# Autodesk Inventor assembly: SHOT_1_002_ShooterAssembly
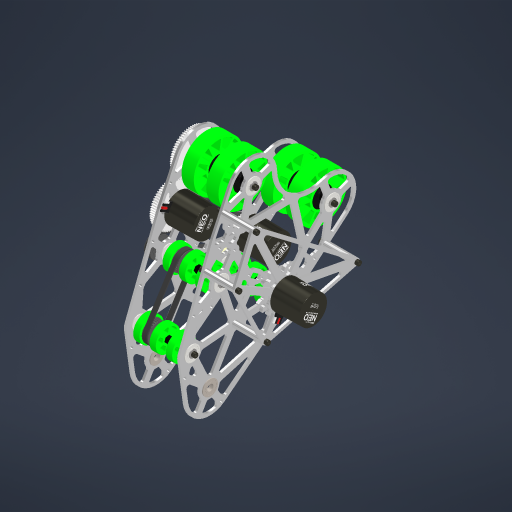
[picture p0: Inventor's stored thumbnail of the model, 512x512]
Saved by Autodesk Inventor 2024.2 (Build 282272000, 272)
## iProperties
Created: 2024-08-07
Part Number: SHOT_1_002_ShooterAssembly
Document SubType Name: Assembly
Designer: Kenji
Mass: 3332.01 g
Surface Area: 7576.03 cm^2
Volume: 1529.69 cm^3
Density: 2.17823 g/cm^3
Author: Kenji
## Documents named in this file (34)
- C:\Users\bobsb\OneDrive\Documents\GitHub\1622-2024-Summer-CAD-A-Thon\Shooter\SHOT_1_002_ShooterAssembly.iam
- C:\Users\bobsb\OneDrive\Documents\GitHub\1622-2024-Summer-CAD-A-Thon\Shooter\SHOT_1_001_ShooterPlate.ipt
- C:\Users\bobsb\OneDrive\Documents\GitHub\1622-2024-Summer-CAD-A-Thon\COTS Library\Motion\Wheels\Compliant Wheels\4in compliant wheels\0.500in hex bore\COTS_am-3462_4indiameter_0.500inhexbore_durometer35A_CompliantWheel.ipt
- C:\Users\bobsb\OneDrive\Documents\GitHub\1622-2024-Summer-CAD-A-Thon\COTS Library\Motion\Bearings\COTS_WCP-0783_1.125ODHexBearing.ipt
- C:\Users\bobsb\OneDrive\Documents\GitHub\1622-2024-Summer-CAD-A-Thon\COTS Library\Motion\Bearings\COTS_WCP-0781_0.5ODCircularFlangedBearing.ipt
- C:\Users\bobsb\OneDrive\Documents\GitHub\1622-2024-Summer-CAD-A-Thon\COTS Library\Motors\COTS_REV-21-1650-V1.1_Neo1.1.ipt
- C:\Users\bobsb\OneDrive\Documents\GitHub\1622-2024-Summer-CAD-A-Thon\COTS Library\Motion\Wheels\Compliant Wheels\2in compliant wheels\0.500in hex bore\COTS_am-3462_2indiameter_0.500inhexbore_durometer35A_CompliantWheel.ipt
- C:\Users\bobsb\OneDrive\Documents\GitHub\1622-2024-Summer-CAD-A-Thon\COTS Library\Fasteners\Bolts\Button-Head\10-32\COTS_92949A265_1-2in long Stainless Steel Button Head Screw.ipt
- C:\Users\bobsb\OneDrive\Documents\GitHub\1622-2024-Summer-CAD-A-Thon\COTS Library\Motion\Pulleys\HTD5M\10mm Wide\COTS_HTD5M10mm24T_WCP-0564.ipt
- C:\Users\bobsb\OneDrive\Documents\GitHub\1622-2024-Summer-CAD-A-Thon\COTS Library\Adapters\COTS_REV-21-1879_8mmKeyTo0.5Hex.ipt
- C:\Users\bobsb\OneDrive\Documents\GitHub\1622-2024-Summer-CAD-A-Thon\COTS Library\Motion\Gears\20DP gears\Aluminum\COTS_WCP-0171_66T.ipt
- C:\Users\bobsb\OneDrive\Documents\GitHub\1622-2024-Summer-CAD-A-Thon\Shooter\SHOT_1_004_66TGear-24TPulley.ipt
- C:\Users\bobsb\OneDrive\Documents\GitHub\1622-2024-Summer-CAD-A-Thon\COTS Library\Motion\Gears\20DP gears\Aluminum\COTS_WCP-0717_54T.ipt
- C:\Users\bobsb\OneDrive\Documents\GitHub\1622-2024-Summer-CAD-A-Thon\Shooter\SHOT_1_005_36TGear-24TPulley.ipt
- C:\Users\bobsb\OneDrive\Documents\GitHub\1622-2024-Summer-CAD-A-Thon\Shooter\SHOT_1_014_Belt3.ipt
- C:\Users\bobsb\OneDrive\Documents\GitHub\1622-2024-Summer-CAD-A-Thon\Shooter\SHOT_1_013_Belt2.ipt
- C:\Users\bobsb\OneDrive\Documents\GitHub\1622-2024-Summer-CAD-A-Thon\Shooter\SHOT_1_012_Belt1.ipt
- C:\Users\bobsb\OneDrive\Documents\GitHub\1622-2024-Summer-CAD-A-Thon\Shooter\SHOT_1_010_Spacer1.ipt
- C:\Users\bobsb\OneDrive\Documents\GitHub\1622-2024-Summer-CAD-A-Thon\Shooter\SHOT_1_011_Spacer2.ipt
- C:\Users\bobsb\OneDrive\Documents\GitHub\1622-2024-Summer-CAD-A-Thon\Shooter\SHOT_1_006_HexShaft1.ipt
- C:\Users\bobsb\OneDrive\Documents\GitHub\1622-2024-Summer-CAD-A-Thon\Shooter\SHOT_1_007_HexShaft2.ipt
- C:\Users\bobsb\OneDrive\Documents\GitHub\1622-2024-Summer-CAD-A-Thon\Shooter\SHOT_1_008_HexShaft3.ipt
- C:\Users\bobsb\OneDrive\Documents\GitHub\1622-2024-Summer-CAD-A-Thon\Shooter\SHOT_1_009_HexShaft4.ipt
- C:\Users\bobsb\OneDrive\Documents\GitHub\1622-2024-Summer-CAD-A-Thon\COTS Library\Fasteners\Bolts\Socket-Head\0.25-20\COTS_91251A539_Black-Oxide Alloy Steel Socket Head Screw (1).ipt
- C:\Users\bobsb\OneDrive\Documents\GitHub\1622-2024-Summer-CAD-A-Thon\COTS Library\Fasteners\Washers\COTS_90107A029_316 Stainless Steel Washer.ipt
- C:\Users\bobsb\OneDrive\Documents\GitHub\1622-2024-Summer-CAD-A-Thon\COTS Library\Fasteners\Bolts\Button-Head\10-32\COTS_92949A267_18-8 Stainless Steel Button Head Hex Drive Screw (1).ipt
- C:\Users\bobsb\OneDrive\Documents\GitHub\1622-2024-Summer-CAD-A-Thon\COTS Library\Fasteners\Washers\COTS_91860A047_Size10Washer.ipt
- C:\Users\bobsb\OneDrive\Documents\GitHub\1622-2024-Summer-CAD-A-Thon\COTS Library\Fasteners\Shaft Collars\COTS_WCP-0799_0.5inchHexShaftCollar.ipt
- C:\Users\bobsb\OneDrive\Documents\GitHub\1622-2024-Summer-CAD-A-Thon\Shooter\SHOT_1_015_PivotCover.ipt
- C:\Users\bobsb\OneDrive\Documents\GitHub\1622-2024-Summer-CAD-A-Thon\Shooter\SHOT_1_016_5DP14TGear.ipt
- C:\Users\bobsb\OneDrive\Documents\GitHub\1622-2024-Summer-CAD-A-Thon\Shooter\SHOT_1_017_Spacer3.ipt
- C:\Users\bobsb\OneDrive\Documents\GitHub\1622-2024-Summer-CAD-A-Thon\Shooter\SHOT_1_0018_Spacer4.ipt
- C:\Users\bobsb\OneDrive\Documents\GitHub\1622-2024-Summer-CAD-A-Thon\Shooter\SHOY_019_Spacer5.ipt
- C:\Users\bobsb\OneDrive\Documents\GitHub\1622-2024-Summer-CAD-A-Thon\COTS Library\Fasteners\Bolts\Button-Head\0.25-20\COTS_0.25-20_ButtonHead_0.5inlong_StainlessSteel_92949A537.ipt
## Components (109 placed, 33 different names)
1. SHOT_1_001_ShooterPlate:1 — Mate:140, Mate:141, Mate:143, Mate:144, Mate:148, Mate:150, Mate:151, Mate:152, Mate:160, Mate:161, Mate:163, Mate:164, Mate:165, Mate:166, Mate:167, Mate:168, Mate:169, Mate:170, Mate:171, Mate:172, Mate:270, Mate:271, Mate:280, Mate:281, Mate:282, Mate:283, Mate:284, Mate:285, Mate:286, Mate:287, Mate:288, Mate:289, Mate:290, Mate:294, Mate:304, Mate:305
2. SHOT_1_001_ShooterPlate:2 — Mate:140, Mate:141, Mate:147, Mate:149, Mate:156, Mate:158, Mate:159, Mate:272, Mate:273, Mate:304, Mate:311, Mate:337, Mate:353, Mate:354, Mate:371, Mate:374, Mate:375, Mate:377, Mate:387, Mate:388, Mate:389, Mate:390, Mate:391, Mate:394, Mate:395, Mate:396, Mate:397
3. COTS_WCP-0783_1.125ODHexBearing:1 — Mate:139, Flush:5, Mate:156, Mate:246
4. COTS_WCP-0783_1.125ODHexBearing:2 — Mate:147, Mate:149, Mate:333, Mate:343
5. COTS_WCP-0783_1.125ODHexBearing:3 — Mate:36, Mate:102, Flush:5, Mate:251
6. COTS_WCP-0783_1.125ODHexBearing:5 — Mate:244, Mate:270, Mate:271, Mate:274, Mate:275
7. COTS_WCP-0783_1.125ODHexBearing:9 — Mate:102, Flush:4, Mate:150, Mate:152, Mate:186, Mate:187
8. COTS_WCP-0783_1.125ODHexBearing:10 — Mate:31, Mate:104, Flush:4, Mate:151, Mate:188, Mate:213
9. COTS_WCP-0783_1.125ODHexBearing:11 — Mate:49, Mate:52, Mate:143, Mate:144, Flush:17, Mate:346
10. COTS_WCP-0783_1.125ODHexBearing:12 — Mate:272, Mate:273, Mate:278
11. COTS_WCP-0781_0.5ODCircularFlangedBearing:1 — Mate:138, Mate:158, Mate:159
12. COTS_WCP-0781_0.5ODCircularFlangedBearing:2 — Mate:138, Mate:160
13. COTS_REV-21-1650-V1.1_Neo1.1:1 — Mate:133, Mate:161, Mate:163, Mate:185, Mate:256, Mate:260, Mate:261, Mate:266
14. COTS_92949A265_1-2in long Stainless Steel Button Head Screw:1 — Mate:165, Mate:168, Mate:185
15. COTS_92949A265_1-2in long Stainless Steel Button Head Screw:2 — Mate:167, Mate:170
16. COTS_92949A265_1-2in long Stainless Steel Button Head Screw:3 — Mate:166, Mate:169
17. COTS_92949A265_1-2in long Stainless Steel Button Head Screw:4 — Mate:164, Mate:171
18. COTS_WCP-0783_1.125ODHexBearing:13 — Mate:148, Mate:305, Mate:306, Mate:342
19. COTS_WCP-0783_1.125ODHexBearing:14 — Mate:308, Mate:311, Mate:337
20. COTS_REV-21-1650-V1.1_Neo1.1:2 — Mate:280, Mate:281, Mate:282, Mate:291, Mate:292, Mate:293, Mate:295
21. COTS_REV-21-1879_8mmKeyTo0.5Hex:1 — Mate:291, Mate:292
22. COTS_92949A265_1-2in long Stainless Steel Button Head Screw:5 — Mate:285, Mate:288
23. COTS_92949A265_1-2in long Stainless Steel Button Head Screw:6 — Mate:286, Mate:290
24. COTS_92949A265_1-2in long Stainless Steel Button Head Screw:7 — Mate:283, Mate:287
25. COTS_92949A265_1-2in long Stainless Steel Button Head Screw:8 — Mate:284, Mate:289
26. SHOT_1_004_66TGear-24TPulley:1 — Mate:133, Mate:172, Flush:6, Mate:198, Mate:257
27. COTS_WCP-0171_66T:1 — Mate:186, Mate:187, Mate:301, Flush:15
28. COTS_HTD5M10mm24T_WCP-0564:1 — Mate:188, Flush:6, Mate:199, Mate:200, Mate:207, Flush:9, Mate:214, Mate:240
29. COTS_WCP-0717_54T:1 — Mate:274, Mate:275, Mate:276, Flush:13, Mate:329, Mate:330
30. SHOT_1_005_36TGear-24TPulley:1 — Mate:293, Mate:294, Mate:296, Flush:16, Mate:318, Mate:319
31. COTS_HTD5M10mm24T_WCP-0564:2 — Mate:320, Mate:331, Mate:339, Mate:340
32. COTS_HTD5M10mm24T_WCP-0564:3 — Flush:16, Mate:307, Mate:317, Mate:326, Flush:18
33. COTS_HTD5M10mm24T_WCP-0564:4 — Mate:255, Mate:314, Mate:321, Mate:335, Mate:336, Mate:338
34. SHOT_1_014_Belt3:1 — Mate:255, Mate:320, Mate:321, Mate:331
35. SHOT_1_013_Belt2:1 — Mate:317, Mate:318, Mate:319
36. SHOT_1_012_Belt1:1 — Mate:198, Mate:199, Mate:200
37. SHOT_1_010_Spacer1:1 — Mate:213, Mate:214
38. SHOT_1_010_Spacer1:2 — Mate:306, Mate:307
39. SHOT_1_006_HexShaft1:1 — Mate:235, Mate:301, Flush:15, Mate:302, Mate:303
40. SHOT_1_007_HexShaft2:1 — Mate:207, Flush:9, Mate:238, Mate:245
41. SHOT_1_009_HexShaft4:1 — Mate:237, Mate:248, Mate:308, Flush:17, Mate:310, Mate:312
42. SHOT_1_006_HexShaft1:2 — Mate:239, Mate:249, Mate:276, Flush:13
43. COTS_91251A539_Black-Oxide Alloy Steel Socket Head Screw (1):1 — Mate:219, Mate:233, Mate:239
44. COTS_91251A539_Black-Oxide Alloy Steel Socket Head Screw (1):2 — Mate:220, Mate:230, Mate:238
45. COTS_91251A539_Black-Oxide Alloy Steel Socket Head Screw (1):3 — Mate:222, Mate:229, Mate:249
46. COTS_91251A539_Black-Oxide Alloy Steel Socket Head Screw (1):4 — Mate:217, Mate:232, Mate:303
47. COTS_91251A539_Black-Oxide Alloy Steel Socket Head Screw (1):5 — Mate:218, Mate:234, Mate:235
48. COTS_91251A539_Black-Oxide Alloy Steel Socket Head Screw (1):6 — Mate:316, Mate:324
49. COTS_91251A539_Black-Oxide Alloy Steel Socket Head Screw (1):7 — Mate:224, Mate:237, Mate:309
50. COTS_91251A539_Black-Oxide Alloy Steel Socket Head Screw (1):8 — Mate:223, Mate:227
51. COTS_91251A539_Black-Oxide Alloy Steel Socket Head Screw (1):9 — Mate:216, Mate:248, Mate:313, Mate:314
52. COTS_91251A539_Black-Oxide Alloy Steel Socket Head Screw (1):10 — Mate:215, Mate:231, Mate:245
53. COTS_90107A029_316 Stainless Steel Washer:1 — Mate:218, Mate:234, Mate:302
54. COTS_90107A029_316 Stainless Steel Washer:2 — Mate:220, Mate:230, Mate:240
55. COTS_90107A029_316 Stainless Steel Washer:3 — Mate:316, Mate:324, Mate:333
56. COTS_90107A029_316 Stainless Steel Washer:4 — Mate:219, Mate:233, Mate:244
57. COTS_90107A029_316 Stainless Steel Washer:5 — Mate:222, Mate:229, Mate:278
58. COTS_90107A029_316 Stainless Steel Washer:6 — Mate:223, Mate:227, Mate:326
59. COTS_90107A029_316 Stainless Steel Washer:7 — Mate:224, Mate:309, Mate:310
60. COTS_90107A029_316 Stainless Steel Washer:8 — Mate:217, Mate:232, Mate:251
61. COTS_90107A029_316 Stainless Steel Washer:9 — Mate:215, Mate:231, Mate:246
62. COTS_90107A029_316 Stainless Steel Washer:10 — Mate:216, Mate:312, Mate:313
63. SHOT_1_011_Spacer2:1 — Mate:256, Mate:257, Mate:267
64. SHOT_1_011_Spacer2:2 — Mate:269, Mate:279, Mate:296
65. COTS_REV-21-1879_8mmKeyTo0.5Hex:2 — Mate:260, Mate:261
66. COTS_92949A267_18-8 Stainless Steel Button Head Hex Drive Screw (1):1 — Mate:263, Mate:265, Mate:266
67. COTS_92949A267_18-8 Stainless Steel Button Head Hex Drive Screw (1):2 — Mate:262, Mate:264, Mate:279, Mate:295
68. COTS_91860A047_Size10Washer:1 — Mate:262, Mate:264, Mate:269
69. COTS_91860A047_Size10Washer:2 — Mate:263, Mate:265, Mate:267
70. COTS_90107A029_316 Stainless Steel Washer:11 — Mate:327, Mate:328, Mate:329, Mate:330
71. COTS_91251A539_Black-Oxide Alloy Steel Socket Head Screw (1):11 — Mate:327, Mate:328
72. COTS_WCP-0799_0.5inchHexShaftCollar:1 — Mate:339, Mate:340, Mate:341
73. COTS_WCP-0799_0.5inchHexShaftCollar:2 — Mate:336, Mate:338
74. COTS_WCP-0799_0.5inchHexShaftCollar:3 — Mate:344, Mate:345
75. COTS_WCP-0799_0.5inchHexShaftCollar:4 — Mate:346, Mate:347
76. SHOT_1_008_HexShaft3:1 — Mate:343, Flush:18
77. SHOT_1_015_PivotCover:3 — Mate:353, Mate:354, Mate:357, Mate:358, Mate:359, Mate:368, Mate:372, Mate:373, Mate:376, Mate:378, Mate:379, Mate:380, Mate:381, Mate:382, Mate:383, Mate:384, Mate:385, Mate:386
78. COTS_REV-21-1650-V1.1_Neo1.1:3 — Mate:357, Mate:358, Mate:359, Mate:360, Mate:361, Mate:362, Mate:367, Mate:369, Mate:398, Mate:401, Mate:402
79. COTS_REV-21-1879_8mmKeyTo0.5Hex:3 — Mate:360, Mate:361
80. COTS_92949A265_1-2in long Stainless Steel Button Head Screw:9 — Mate:362, Mate:403
81. SHOT_1_017_Spacer3:1 — Mate:367, Mate:368, Mate:399
82. SHOT_1_0018_Spacer4:1 — Mate:369, Mate:400
83. SHOY_019_Spacer5:1 — Mate:377, Mate:378
84. SHOY_019_Spacer5:2 — Mate:375, Mate:376, Mate:397
85. SHOY_019_Spacer5:3 — Mate:371, Mate:372
86. SHOY_019_Spacer5:4 — Mate:373, Mate:374
87. COTS_91251A539_Black-Oxide Alloy Steel Socket Head Screw (1):13 — Mate:382, Mate:384
88. COTS_91251A539_Black-Oxide Alloy Steel Socket Head Screw (1):14 — Mate:388, Mate:390
89. COTS_91251A539_Black-Oxide Alloy Steel Socket Head Screw (1):15 — Mate:391, Mate:394
90. COTS_91251A539_Black-Oxide Alloy Steel Socket Head Screw (1):16 — Mate:387, Mate:389
91. COTS_91251A539_Black-Oxide Alloy Steel Socket Head Screw (1):17 — Mate:379, Mate:385
92. COTS_91251A539_Black-Oxide Alloy Steel Socket Head Screw (1):18 — Mate:380, Mate:386
93. COTS_91251A539_Black-Oxide Alloy Steel Socket Head Screw (1):19 — Mate:381, Mate:383
94. COTS_0.25-20_ButtonHead_0.5inlong_StainlessSteel_92949A537:1 — Mate:395, Mate:396
95. SHOT_1_016_5DP14TGear:2 — Mate:398, Mate:399, Mate:400
96. COTS_90107A029_316 Stainless Steel Washer:12 — Mate:401, Mate:402, Mate:403
97. COTS_am-3462_4indiameter_0.500inhexbore_durometer35A_CompliantWheel:4 — Mate:36, Flush:3
98. COTS_am-3462_4indiameter_0.500inhexbore_durometer35A_CompliantWheel:1 — Mate:31, Flush:3, Mate:104
99. COTS_am-3462_4indiameter_0.500inhexbore_durometer35A_CompliantWheel:5
100. COTS_am-3462_4indiameter_0.500inhexbore_durometer35A_CompliantWheel:6 — Mate:139
101. COTS_am-3462_2indiameter_0.500inhexbore_durometer35A_CompliantWheel:1 — Flush:1, Flush:2
102. COTS_am-3462_2indiameter_0.500inhexbore_durometer35A_CompliantWheel:6 — Flush:2, Mate:341, Mate:342, Mate:344, Mate:345
103. COTS_am-3462_2indiameter_0.500inhexbore_durometer35A_CompliantWheel:2 — Mate:49, Flush:1, Mate:52, Mate:335, Mate:347
104. COTS_am-3462_2indiameter_0.500inhexbore_durometer35A_CompliantWheel:7
105. COTS_am-3462_2indiameter_0.500inhexbore_durometer35A_CompliantWheel:8
106. COTS_am-3462_2indiameter_0.500inhexbore_durometer35A_CompliantWheel:9
107. COTS_am-3462_2indiameter_0.500inhexbore_durometer35A_CompliantWheel:10
108. COTS_am-3462_2indiameter_0.500inhexbore_durometer35A_CompliantWheel:11
109. COTS_am-3462_2indiameter_0.500inhexbore_durometer35A_CompliantWheel:12
## Component patterns: (2 elements, first: COTS_am-3462_4indiameter_0.500inhexbore_durometer35A_CompliantWheel:4 + COTS_am-3462_4indiameter_0.500inhexbore_durometer35A_CompliantWheel:1), (3 elements, first: COTS_am-3462_2indiameter_0.500inhexbore_durometer35A_CompliantWheel:1 + COTS_am-3462_2indiameter_0.500inhexbore_durometer35A_CompliantWheel:6 + COTS_am-3462_2indiameter_0.500inhexbore_durometer35A_CompliantWheel:2)
## Relationships (204: Mate 192, Flush 12)
- Mate:31: COTS_WCP-0783_1.125ODHexBearing:10 ↔ COTS_am-3462_4indiameter_0.500inhexbore_durometer35A_CompliantWheel:1
- Mate:36: COTS_WCP-0783_1.125ODHexBearing:3 ↔ COTS_am-3462_4indiameter_0.500inhexbore_durometer35A_CompliantWheel:4
- Mate:49: COTS_WCP-0783_1.125ODHexBearing:11 ↔ COTS_am-3462_2indiameter_0.500inhexbore_durometer35A_CompliantWheel:2
- Flush:1: COTS_am-3462_2indiameter_0.500inhexbore_durometer35A_CompliantWheel:1 ↔ COTS_am-3462_2indiameter_0.500inhexbore_durometer35A_CompliantWheel:2
- Flush:2: COTS_am-3462_2indiameter_0.500inhexbore_durometer35A_CompliantWheel:1 ↔ COTS_am-3462_2indiameter_0.500inhexbore_durometer35A_CompliantWheel:6
- Mate:52 (12.7 mm): COTS_WCP-0783_1.125ODHexBearing:11 ↔ COTS_am-3462_2indiameter_0.500inhexbore_durometer35A_CompliantWheel:2
- Mate:102: COTS_WCP-0783_1.125ODHexBearing:3 ↔ COTS_WCP-0783_1.125ODHexBearing:9
- Flush:3: COTS_am-3462_4indiameter_0.500inhexbore_durometer35A_CompliantWheel:4 ↔ COTS_am-3462_4indiameter_0.500inhexbore_durometer35A_CompliantWheel:1
- Mate:104 (12.7 mm): COTS_WCP-0783_1.125ODHexBearing:10 ↔ COTS_am-3462_4indiameter_0.500inhexbore_durometer35A_CompliantWheel:1
- Mate:133: COTS_REV-21-1650-V1.1_Neo1.1:1 ↔ SHOT_1_004_66TGear-24TPulley:1
- Mate:138: COTS_WCP-0781_0.5ODCircularFlangedBearing:1 ↔ COTS_WCP-0781_0.5ODCircularFlangedBearing:2
- Mate:139: COTS_WCP-0783_1.125ODHexBearing:1 ↔ COTS_am-3462_4indiameter_0.500inhexbore_durometer35A_CompliantWheel:6
- Flush:4: COTS_WCP-0783_1.125ODHexBearing:9 ↔ COTS_WCP-0783_1.125ODHexBearing:10
- Flush:5: COTS_WCP-0783_1.125ODHexBearing:1 ↔ COTS_WCP-0783_1.125ODHexBearing:3
- Mate:140: SHOT_1_001_ShooterPlate:1 ↔ SHOT_1_001_ShooterPlate:2
- Mate:141: SHOT_1_001_ShooterPlate:1 ↔ SHOT_1_001_ShooterPlate:2
- Mate:143: SHOT_1_001_ShooterPlate:1 ↔ COTS_WCP-0783_1.125ODHexBearing:11
- Mate:144: SHOT_1_001_ShooterPlate:1 ↔ COTS_WCP-0783_1.125ODHexBearing:11
- Mate:147: SHOT_1_001_ShooterPlate:2 ↔ COTS_WCP-0783_1.125ODHexBearing:2
- Mate:148: SHOT_1_001_ShooterPlate:1 ↔ COTS_WCP-0783_1.125ODHexBearing:13
- Mate:149: SHOT_1_001_ShooterPlate:2 ↔ COTS_WCP-0783_1.125ODHexBearing:2
- Mate:150: SHOT_1_001_ShooterPlate:1 ↔ COTS_WCP-0783_1.125ODHexBearing:9
- Mate:151: SHOT_1_001_ShooterPlate:1 ↔ COTS_WCP-0783_1.125ODHexBearing:10
- Mate:152: SHOT_1_001_ShooterPlate:1 ↔ COTS_WCP-0783_1.125ODHexBearing:9
- Mate:156: SHOT_1_001_ShooterPlate:2 ↔ COTS_WCP-0783_1.125ODHexBearing:1
- Mate:158: SHOT_1_001_ShooterPlate:2 ↔ COTS_WCP-0781_0.5ODCircularFlangedBearing:1
- Mate:159: SHOT_1_001_ShooterPlate:2 ↔ COTS_WCP-0781_0.5ODCircularFlangedBearing:1
- Mate:160: SHOT_1_001_ShooterPlate:1 ↔ COTS_WCP-0781_0.5ODCircularFlangedBearing:2
- Mate:161: SHOT_1_001_ShooterPlate:1 ↔ COTS_REV-21-1650-V1.1_Neo1.1:1
- Mate:163: SHOT_1_001_ShooterPlate:1 ↔ COTS_REV-21-1650-V1.1_Neo1.1:1
- Mate:164: SHOT_1_001_ShooterPlate:1 ↔ COTS_92949A265_1-2in long Stainless Steel Button Head Screw:4
- Mate:165: SHOT_1_001_ShooterPlate:1 ↔ COTS_92949A265_1-2in long Stainless Steel Button Head Screw:1
- Mate:166: SHOT_1_001_ShooterPlate:1 ↔ COTS_92949A265_1-2in long Stainless Steel Button Head Screw:3
- Mate:167: SHOT_1_001_ShooterPlate:1 ↔ COTS_92949A265_1-2in long Stainless Steel Button Head Screw:2
- Mate:168: SHOT_1_001_ShooterPlate:1 ↔ COTS_92949A265_1-2in long Stainless Steel Button Head Screw:1
- Mate:169: SHOT_1_001_ShooterPlate:1 ↔ COTS_92949A265_1-2in long Stainless Steel Button Head Screw:3
- Mate:170: SHOT_1_001_ShooterPlate:1 ↔ COTS_92949A265_1-2in long Stainless Steel Button Head Screw:2
- Mate:171: SHOT_1_001_ShooterPlate:1 ↔ COTS_92949A265_1-2in long Stainless Steel Button Head Screw:4
- Mate:172: SHOT_1_001_ShooterPlate:1 ↔ SHOT_1_004_66TGear-24TPulley:1
- Mate:185: COTS_REV-21-1650-V1.1_Neo1.1:1 ↔ COTS_92949A265_1-2in long Stainless Steel Button Head Screw:1
- Mate:186: COTS_WCP-0783_1.125ODHexBearing:9 ↔ COTS_WCP-0171_66T:1
- Mate:187: COTS_WCP-0783_1.125ODHexBearing:9 ↔ COTS_WCP-0171_66T:1
- Mate:188: COTS_WCP-0783_1.125ODHexBearing:10 ↔ COTS_HTD5M10mm24T_WCP-0564:1
- Flush:6: SHOT_1_004_66TGear-24TPulley:1 ↔ COTS_HTD5M10mm24T_WCP-0564:1
- Mate:198: SHOT_1_004_66TGear-24TPulley:1 ↔ SHOT_1_012_Belt1:1
- Mate:199: COTS_HTD5M10mm24T_WCP-0564:1 ↔ SHOT_1_012_Belt1:1
- Mate:200: COTS_HTD5M10mm24T_WCP-0564:1 ↔ SHOT_1_012_Belt1:1
- Mate:207: COTS_HTD5M10mm24T_WCP-0564:1 ↔ SHOT_1_007_HexShaft2:1
- Flush:9: COTS_HTD5M10mm24T_WCP-0564:1 ↔ SHOT_1_007_HexShaft2:1
- Mate:213: COTS_WCP-0783_1.125ODHexBearing:10 ↔ SHOT_1_010_Spacer1:1
- Mate:214: COTS_HTD5M10mm24T_WCP-0564:1 ↔ SHOT_1_010_Spacer1:1
- Mate:215: COTS_91251A539_Black-Oxide Alloy Steel Socket Head Screw (1):10 ↔ COTS_90107A029_316 Stainless Steel Washer:9
- Mate:216: COTS_91251A539_Black-Oxide Alloy Steel Socket Head Screw (1):9 ↔ COTS_90107A029_316 Stainless Steel Washer:10
- Mate:217: COTS_91251A539_Black-Oxide Alloy Steel Socket Head Screw (1):4 ↔ COTS_90107A029_316 Stainless Steel Washer:8
- Mate:218: COTS_91251A539_Black-Oxide Alloy Steel Socket Head Screw (1):5 ↔ COTS_90107A029_316 Stainless Steel Washer:1
- Mate:219: COTS_91251A539_Black-Oxide Alloy Steel Socket Head Screw (1):1 ↔ COTS_90107A029_316 Stainless Steel Washer:4
- Mate:220: COTS_91251A539_Black-Oxide Alloy Steel Socket Head Screw (1):2 ↔ COTS_90107A029_316 Stainless Steel Washer:2
- Mate:222: COTS_91251A539_Black-Oxide Alloy Steel Socket Head Screw (1):3 ↔ COTS_90107A029_316 Stainless Steel Washer:5
- Mate:223: COTS_91251A539_Black-Oxide Alloy Steel Socket Head Screw (1):8 ↔ COTS_90107A029_316 Stainless Steel Washer:6
- Mate:224: COTS_91251A539_Black-Oxide Alloy Steel Socket Head Screw (1):7 ↔ COTS_90107A029_316 Stainless Steel Washer:7
- Mate:227: COTS_91251A539_Black-Oxide Alloy Steel Socket Head Screw (1):8 ↔ COTS_90107A029_316 Stainless Steel Washer:6
- Mate:229: COTS_91251A539_Black-Oxide Alloy Steel Socket Head Screw (1):3 ↔ COTS_90107A029_316 Stainless Steel Washer:5
- Mate:230: COTS_91251A539_Black-Oxide Alloy Steel Socket Head Screw (1):2 ↔ COTS_90107A029_316 Stainless Steel Washer:2
- Mate:231: COTS_91251A539_Black-Oxide Alloy Steel Socket Head Screw (1):10 ↔ COTS_90107A029_316 Stainless Steel Washer:9
- Mate:232: COTS_91251A539_Black-Oxide Alloy Steel Socket Head Screw (1):4 ↔ COTS_90107A029_316 Stainless Steel Washer:8
- Mate:233: COTS_91251A539_Black-Oxide Alloy Steel Socket Head Screw (1):1 ↔ COTS_90107A029_316 Stainless Steel Washer:4
- Mate:234: COTS_91251A539_Black-Oxide Alloy Steel Socket Head Screw (1):5 ↔ COTS_90107A029_316 Stainless Steel Washer:1
- Mate:235: SHOT_1_006_HexShaft1:1 ↔ COTS_91251A539_Black-Oxide Alloy Steel Socket Head Screw (1):5
- Mate:237: SHOT_1_009_HexShaft4:1 ↔ COTS_91251A539_Black-Oxide Alloy Steel Socket Head Screw (1):7
- Mate:238: SHOT_1_007_HexShaft2:1 ↔ COTS_91251A539_Black-Oxide Alloy Steel Socket Head Screw (1):2
- Mate:239: SHOT_1_006_HexShaft1:2 ↔ COTS_91251A539_Black-Oxide Alloy Steel Socket Head Screw (1):1
- Mate:240: COTS_HTD5M10mm24T_WCP-0564:1 ↔ COTS_90107A029_316 Stainless Steel Washer:2
- Mate:244: COTS_WCP-0783_1.125ODHexBearing:5 ↔ COTS_90107A029_316 Stainless Steel Washer:4
- Mate:245: SHOT_1_007_HexShaft2:1 ↔ COTS_91251A539_Black-Oxide Alloy Steel Socket Head Screw (1):10
- Mate:246: COTS_WCP-0783_1.125ODHexBearing:1 ↔ COTS_90107A029_316 Stainless Steel Washer:9
- Mate:248: SHOT_1_009_HexShaft4:1 ↔ COTS_91251A539_Black-Oxide Alloy Steel Socket Head Screw (1):9
- Mate:249: SHOT_1_006_HexShaft1:2 ↔ COTS_91251A539_Black-Oxide Alloy Steel Socket Head Screw (1):3
- Mate:251: COTS_WCP-0783_1.125ODHexBearing:3 ↔ COTS_90107A029_316 Stainless Steel Washer:8
- Mate:255: COTS_HTD5M10mm24T_WCP-0564:4 ↔ SHOT_1_014_Belt3:1
- Mate:256: COTS_REV-21-1650-V1.1_Neo1.1:1 ↔ SHOT_1_011_Spacer2:1
- Mate:257: SHOT_1_004_66TGear-24TPulley:1 ↔ SHOT_1_011_Spacer2:1
- Mate:260: COTS_REV-21-1650-V1.1_Neo1.1:1 ↔ COTS_REV-21-1879_8mmKeyTo0.5Hex:2
- Mate:261: COTS_REV-21-1650-V1.1_Neo1.1:1 ↔ COTS_REV-21-1879_8mmKeyTo0.5Hex:2
- Mate:262: COTS_92949A267_18-8 Stainless Steel Button Head Hex Drive Screw (1):2 ↔ COTS_91860A047_Size10Washer:1
- Mate:263: COTS_92949A267_18-8 Stainless Steel Button Head Hex Drive Screw (1):1 ↔ COTS_91860A047_Size10Washer:2
- Mate:264: COTS_92949A267_18-8 Stainless Steel Button Head Hex Drive Screw (1):2 ↔ COTS_91860A047_Size10Washer:1
- Mate:265: COTS_92949A267_18-8 Stainless Steel Button Head Hex Drive Screw (1):1 ↔ COTS_91860A047_Size10Washer:2
- Mate:266: COTS_REV-21-1650-V1.1_Neo1.1:1 ↔ COTS_92949A267_18-8 Stainless Steel Button Head Hex Drive Screw (1):1
- Mate:267: SHOT_1_011_Spacer2:1 ↔ COTS_91860A047_Size10Washer:2
- Mate:269: SHOT_1_011_Spacer2:2 ↔ COTS_91860A047_Size10Washer:1
- Mate:270: SHOT_1_001_ShooterPlate:1 ↔ COTS_WCP-0783_1.125ODHexBearing:5
- Mate:271: SHOT_1_001_ShooterPlate:1 ↔ COTS_WCP-0783_1.125ODHexBearing:5
- Mate:272: SHOT_1_001_ShooterPlate:2 ↔ COTS_WCP-0783_1.125ODHexBearing:12
- Mate:273: SHOT_1_001_ShooterPlate:2 ↔ COTS_WCP-0783_1.125ODHexBearing:12
- Mate:274: COTS_WCP-0783_1.125ODHexBearing:5 ↔ COTS_WCP-0717_54T:1
- Mate:275: COTS_WCP-0783_1.125ODHexBearing:5 ↔ COTS_WCP-0717_54T:1
- Mate:276: COTS_WCP-0717_54T:1 ↔ SHOT_1_006_HexShaft1:2
- Flush:13: COTS_WCP-0717_54T:1 ↔ SHOT_1_006_HexShaft1:2
- Mate:278: COTS_WCP-0783_1.125ODHexBearing:12 ↔ COTS_90107A029_316 Stainless Steel Washer:5
- Mate:279: SHOT_1_011_Spacer2:2 ↔ COTS_92949A267_18-8 Stainless Steel Button Head Hex Drive Screw (1):2
- Mate:280: SHOT_1_001_ShooterPlate:1 ↔ COTS_REV-21-1650-V1.1_Neo1.1:2
- Mate:281: SHOT_1_001_ShooterPlate:1 ↔ COTS_REV-21-1650-V1.1_Neo1.1:2
- Mate:282: SHOT_1_001_ShooterPlate:1 ↔ COTS_REV-21-1650-V1.1_Neo1.1:2
- Mate:283: SHOT_1_001_ShooterPlate:1 ↔ COTS_92949A265_1-2in long Stainless Steel Button Head Screw:7
- Mate:284: SHOT_1_001_ShooterPlate:1 ↔ COTS_92949A265_1-2in long Stainless Steel Button Head Screw:8
- Mate:285: SHOT_1_001_ShooterPlate:1 ↔ COTS_92949A265_1-2in long Stainless Steel Button Head Screw:5
- Mate:286: SHOT_1_001_ShooterPlate:1 ↔ COTS_92949A265_1-2in long Stainless Steel Button Head Screw:6
- Mate:287: SHOT_1_001_ShooterPlate:1 ↔ COTS_92949A265_1-2in long Stainless Steel Button Head Screw:7
- Mate:288: SHOT_1_001_ShooterPlate:1 ↔ COTS_92949A265_1-2in long Stainless Steel Button Head Screw:5
- Mate:289: SHOT_1_001_ShooterPlate:1 ↔ COTS_92949A265_1-2in long Stainless Steel Button Head Screw:8
- Mate:290: SHOT_1_001_ShooterPlate:1 ↔ COTS_92949A265_1-2in long Stainless Steel Button Head Screw:6
- Mate:291: COTS_REV-21-1650-V1.1_Neo1.1:2 ↔ COTS_REV-21-1879_8mmKeyTo0.5Hex:1
- Mate:292: COTS_REV-21-1650-V1.1_Neo1.1:2 ↔ COTS_REV-21-1879_8mmKeyTo0.5Hex:1
- Mate:293: COTS_REV-21-1650-V1.1_Neo1.1:2 ↔ SHOT_1_005_36TGear-24TPulley:1
- Mate:294: SHOT_1_001_ShooterPlate:1 ↔ SHOT_1_005_36TGear-24TPulley:1
- Mate:295: COTS_REV-21-1650-V1.1_Neo1.1:2 ↔ COTS_92949A267_18-8 Stainless Steel Button Head Hex Drive Screw (1):2
- Mate:296: SHOT_1_005_36TGear-24TPulley:1 ↔ SHOT_1_011_Spacer2:2
- Mate:301: COTS_WCP-0171_66T:1 ↔ SHOT_1_006_HexShaft1:1
- Flush:15: COTS_WCP-0171_66T:1 ↔ SHOT_1_006_HexShaft1:1
- Mate:302: SHOT_1_006_HexShaft1:1 ↔ COTS_90107A029_316 Stainless Steel Washer:1
- Mate:303: SHOT_1_006_HexShaft1:1 ↔ COTS_91251A539_Black-Oxide Alloy Steel Socket Head Screw (1):4
- Mate:304 (104.775 mm): SHOT_1_001_ShooterPlate:1 ↔ SHOT_1_001_ShooterPlate:2
- Mate:305: SHOT_1_001_ShooterPlate:1 ↔ COTS_WCP-0783_1.125ODHexBearing:13
- Flush:16: SHOT_1_005_36TGear-24TPulley:1 ↔ COTS_HTD5M10mm24T_WCP-0564:3
- Mate:306: COTS_WCP-0783_1.125ODHexBearing:13 ↔ SHOT_1_010_Spacer1:2
- Mate:307: COTS_HTD5M10mm24T_WCP-0564:3 ↔ SHOT_1_010_Spacer1:2
- Mate:308: COTS_WCP-0783_1.125ODHexBearing:14 ↔ SHOT_1_009_HexShaft4:1
- Flush:17: COTS_WCP-0783_1.125ODHexBearing:11 ↔ SHOT_1_009_HexShaft4:1
- Mate:309: COTS_91251A539_Black-Oxide Alloy Steel Socket Head Screw (1):7 ↔ COTS_90107A029_316 Stainless Steel Washer:7
- Mate:310: SHOT_1_009_HexShaft4:1 ↔ COTS_90107A029_316 Stainless Steel Washer:7
- Mate:311: SHOT_1_001_ShooterPlate:2 ↔ COTS_WCP-0783_1.125ODHexBearing:14
- Mate:312: SHOT_1_009_HexShaft4:1 ↔ COTS_90107A029_316 Stainless Steel Washer:10
- Mate:313: COTS_91251A539_Black-Oxide Alloy Steel Socket Head Screw (1):9 ↔ COTS_90107A029_316 Stainless Steel Washer:10
- Mate:314: COTS_HTD5M10mm24T_WCP-0564:4 ↔ COTS_91251A539_Black-Oxide Alloy Steel Socket Head Screw (1):9
- Mate:316: COTS_91251A539_Black-Oxide Alloy Steel Socket Head Screw (1):6 ↔ COTS_90107A029_316 Stainless Steel Washer:3
- Mate:317: COTS_HTD5M10mm24T_WCP-0564:3 ↔ SHOT_1_013_Belt2:1
- Mate:318: SHOT_1_005_36TGear-24TPulley:1 ↔ SHOT_1_013_Belt2:1
- Mate:319: SHOT_1_005_36TGear-24TPulley:1 ↔ SHOT_1_013_Belt2:1
- Mate:320: COTS_HTD5M10mm24T_WCP-0564:2 ↔ SHOT_1_014_Belt3:1
- Mate:321: COTS_HTD5M10mm24T_WCP-0564:4 ↔ SHOT_1_014_Belt3:1
- Mate:324: COTS_91251A539_Black-Oxide Alloy Steel Socket Head Screw (1):6 ↔ COTS_90107A029_316 Stainless Steel Washer:3
- Mate:326: COTS_HTD5M10mm24T_WCP-0564:3 ↔ COTS_90107A029_316 Stainless Steel Washer:6
- Mate:327: COTS_90107A029_316 Stainless Steel Washer:11 ↔ COTS_91251A539_Black-Oxide Alloy Steel Socket Head Screw (1):11
- Mate:328: COTS_90107A029_316 Stainless Steel Washer:11 ↔ COTS_91251A539_Black-Oxide Alloy Steel Socket Head Screw (1):11
- Mate:329: COTS_WCP-0717_54T:1 ↔ COTS_90107A029_316 Stainless Steel Washer:11
- Mate:330: COTS_WCP-0717_54T:1 ↔ COTS_90107A029_316 Stainless Steel Washer:11
- Mate:331: COTS_HTD5M10mm24T_WCP-0564:2 ↔ SHOT_1_014_Belt3:1
- Mate:333: COTS_WCP-0783_1.125ODHexBearing:2 ↔ COTS_90107A029_316 Stainless Steel Washer:3
- Mate:335: COTS_HTD5M10mm24T_WCP-0564:4 ↔ COTS_am-3462_2indiameter_0.500inhexbore_durometer35A_CompliantWheel:2
- Mate:336: COTS_HTD5M10mm24T_WCP-0564:4 ↔ COTS_WCP-0799_0.5inchHexShaftCollar:2
- Mate:337: SHOT_1_001_ShooterPlate:2 ↔ COTS_WCP-0783_1.125ODHexBearing:14
- Mate:338: COTS_HTD5M10mm24T_WCP-0564:4 ↔ COTS_WCP-0799_0.5inchHexShaftCollar:2
- Mate:339: COTS_HTD5M10mm24T_WCP-0564:2 ↔ COTS_WCP-0799_0.5inchHexShaftCollar:1
- Mate:340: COTS_HTD5M10mm24T_WCP-0564:2 ↔ COTS_WCP-0799_0.5inchHexShaftCollar:1
- Mate:341: COTS_WCP-0799_0.5inchHexShaftCollar:1 ↔ COTS_am-3462_2indiameter_0.500inhexbore_durometer35A_CompliantWheel:6
- Mate:342: COTS_WCP-0783_1.125ODHexBearing:13 ↔ COTS_am-3462_2indiameter_0.500inhexbore_durometer35A_CompliantWheel:6
- Mate:343: COTS_WCP-0783_1.125ODHexBearing:2 ↔ SHOT_1_008_HexShaft3:1
- Flush:18: COTS_HTD5M10mm24T_WCP-0564:3 ↔ SHOT_1_008_HexShaft3:1
- Mate:344: COTS_WCP-0799_0.5inchHexShaftCollar:3 ↔ COTS_am-3462_2indiameter_0.500inhexbore_durometer35A_CompliantWheel:6
- Mate:345: COTS_WCP-0799_0.5inchHexShaftCollar:3 ↔ COTS_am-3462_2indiameter_0.500inhexbore_durometer35A_CompliantWheel:6
- Mate:346: COTS_WCP-0783_1.125ODHexBearing:11 ↔ COTS_WCP-0799_0.5inchHexShaftCollar:4
- Mate:347: COTS_WCP-0799_0.5inchHexShaftCollar:4 ↔ COTS_am-3462_2indiameter_0.500inhexbore_durometer35A_CompliantWheel:2
- Mate:353: SHOT_1_001_ShooterPlate:2 ↔ SHOT_1_015_PivotCover:3
- Mate:354: SHOT_1_001_ShooterPlate:2 ↔ SHOT_1_015_PivotCover:3
- Mate:357: SHOT_1_015_PivotCover:3 ↔ COTS_REV-21-1650-V1.1_Neo1.1:3
- Mate:358: SHOT_1_015_PivotCover:3 ↔ COTS_REV-21-1650-V1.1_Neo1.1:3
- Mate:359: SHOT_1_015_PivotCover:3 ↔ COTS_REV-21-1650-V1.1_Neo1.1:3
- Mate:360: COTS_REV-21-1650-V1.1_Neo1.1:3 ↔ COTS_REV-21-1879_8mmKeyTo0.5Hex:3
- Mate:361: COTS_REV-21-1650-V1.1_Neo1.1:3 ↔ COTS_REV-21-1879_8mmKeyTo0.5Hex:3
- Mate:362: COTS_REV-21-1650-V1.1_Neo1.1:3 ↔ COTS_92949A265_1-2in long Stainless Steel Button Head Screw:9
- Mate:367: COTS_REV-21-1650-V1.1_Neo1.1:3 ↔ SHOT_1_017_Spacer3:1
- Mate:368: SHOT_1_015_PivotCover:3 ↔ SHOT_1_017_Spacer3:1
- Mate:369: COTS_REV-21-1650-V1.1_Neo1.1:3 ↔ SHOT_1_0018_Spacer4:1
- Mate:371: SHOT_1_001_ShooterPlate:2 ↔ SHOY_019_Spacer5:3
- Mate:372: SHOT_1_015_PivotCover:3 ↔ SHOY_019_Spacer5:3
- Mate:373: SHOT_1_015_PivotCover:3 ↔ SHOY_019_Spacer5:4
- Mate:374: SHOT_1_001_ShooterPlate:2 ↔ SHOY_019_Spacer5:4
- Mate:375: SHOT_1_001_ShooterPlate:2 ↔ SHOY_019_Spacer5:2
- Mate:376: SHOT_1_015_PivotCover:3 ↔ SHOY_019_Spacer5:2
- Mate:377: SHOT_1_001_ShooterPlate:2 ↔ SHOY_019_Spacer5:1
- Mate:378: SHOT_1_015_PivotCover:3 ↔ SHOY_019_Spacer5:1
- Mate:379: SHOT_1_015_PivotCover:3 ↔ COTS_91251A539_Black-Oxide Alloy Steel Socket Head Screw (1):17
- Mate:380: SHOT_1_015_PivotCover:3 ↔ COTS_91251A539_Black-Oxide Alloy Steel Socket Head Screw (1):18
- Mate:381: SHOT_1_015_PivotCover:3 ↔ COTS_91251A539_Black-Oxide Alloy Steel Socket Head Screw (1):19
- Mate:382: SHOT_1_015_PivotCover:3 ↔ COTS_91251A539_Black-Oxide Alloy Steel Socket Head Screw (1):13
- Mate:383: SHOT_1_015_PivotCover:3 ↔ COTS_91251A539_Black-Oxide Alloy Steel Socket Head Screw (1):19
- Mate:384: SHOT_1_015_PivotCover:3 ↔ COTS_91251A539_Black-Oxide Alloy Steel Socket Head Screw (1):13
- Mate:385: SHOT_1_015_PivotCover:3 ↔ COTS_91251A539_Black-Oxide Alloy Steel Socket Head Screw (1):17
- Mate:386: SHOT_1_015_PivotCover:3 ↔ COTS_91251A539_Black-Oxide Alloy Steel Socket Head Screw (1):18
- Mate:387: SHOT_1_001_ShooterPlate:2 ↔ COTS_91251A539_Black-Oxide Alloy Steel Socket Head Screw (1):16
- Mate:388: SHOT_1_001_ShooterPlate:2 ↔ COTS_91251A539_Black-Oxide Alloy Steel Socket Head Screw (1):14
- Mate:389: SHOT_1_001_ShooterPlate:2 ↔ COTS_91251A539_Black-Oxide Alloy Steel Socket Head Screw (1):16
- Mate:390: SHOT_1_001_ShooterPlate:2 ↔ COTS_91251A539_Black-Oxide Alloy Steel Socket Head Screw (1):14
- Mate:391: SHOT_1_001_ShooterPlate:2 ↔ COTS_91251A539_Black-Oxide Alloy Steel Socket Head Screw (1):15
- Mate:394: SHOT_1_001_ShooterPlate:2 ↔ COTS_91251A539_Black-Oxide Alloy Steel Socket Head Screw (1):15
- Mate:395: SHOT_1_001_ShooterPlate:2 ↔ COTS_0.25-20_ButtonHead_0.5inlong_StainlessSteel_92949A537:1
- Mate:396: SHOT_1_001_ShooterPlate:2 ↔ COTS_0.25-20_ButtonHead_0.5inlong_StainlessSteel_92949A537:1
- Mate:397: SHOT_1_001_ShooterPlate:2 ↔ SHOY_019_Spacer5:2
- Mate:398: COTS_REV-21-1650-V1.1_Neo1.1:3 ↔ SHOT_1_016_5DP14TGear:2
- Mate:399: SHOT_1_017_Spacer3:1 ↔ SHOT_1_016_5DP14TGear:2
- Mate:400: SHOT_1_0018_Spacer4:1 ↔ SHOT_1_016_5DP14TGear:2
- Mate:401: COTS_REV-21-1650-V1.1_Neo1.1:3 ↔ COTS_90107A029_316 Stainless Steel Washer:12
- Mate:402: COTS_REV-21-1650-V1.1_Neo1.1:3 ↔ COTS_90107A029_316 Stainless Steel Washer:12
- Mate:403: COTS_92949A265_1-2in long Stainless Steel Button Head Screw:9 ↔ COTS_90107A029_316 Stainless Steel Washer:12
